# Autodesk Inventor assembly: Intake new robot
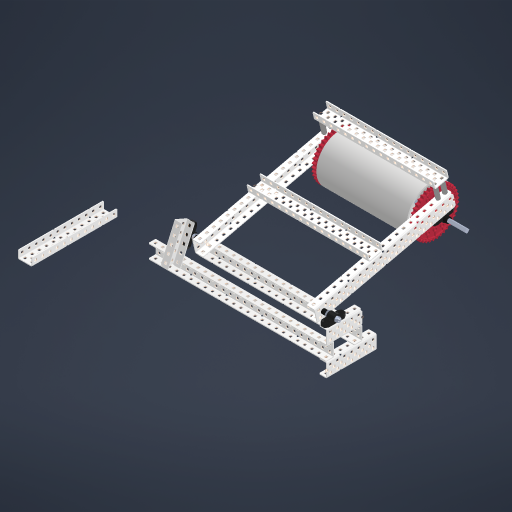
[picture p0: Inventor's stored thumbnail of the model, 512x512]
Saved by Autodesk Inventor 2023.4 (Build 274418000, 418)
## iProperties
Created: 2023-12-04
Part Number: Intake new robot
Document SubType Name: Assembly
Designer: diego
Author: diego
## Documents named in this file (26)
- C:\Users\diego\OneDrive\Documents\GitHub\2024-599Z\2024-599Z\Cad\Intake new robot.iam
- C:\Users\diego\OneDrive\Documents\GitHub\2024-599Z\2024-599Z\Cad\VEX-CAD-Inventor-1.4.0\Structure\C Channel\Aluminum 1x2x1\Alu C 1x2x1x20.ipt
- C:\Users\diego\OneDrive\Documents\GitHub\2024-599Z\2024-599Z\Cad\VEX-CAD-Inventor-1.4.0\Structure\C Channel\Aluminum 1x2x1\Alu C 1x2x1x5.ipt
- C:\Users\diego\OneDrive\Documents\GitHub\2024-599Z\2024-599Z\Cad\VEX-CAD-Inventor-1.4.0\Motion\Shaft HS\HS Pillow Bearing Block.ipt
- C:\Users\diego\OneDrive\Documents\GitHub\2024-599Z\2024-599Z\Cad\VEX-CAD-Inventor-1.4.0\Motion\Spacers\Spacer Plastic.ipt
- C:\Users\diego\OneDrive\Documents\GitHub\2024-599Z\2024-599Z\Cad\VEX-CAD-Inventor-1.4.0\Structure\Hardware\Nut Keps.ipt
- C:\Users\diego\OneDrive\Documents\GitHub\2024-599Z\2024-599Z\Cad\VEX-CAD-Inventor-1.4.0\Structure\Hardware\Screw Steel - Star\SScrew Star Smooth 1.250.ipt
- C:\Users\diego\OneDrive\Documents\GitHub\2024-599Z\2024-599Z\Cad\VEX-CAD-Inventor-1.4.0\Structure\Hardware\Screw Steel - Star.ipt
- C:\Users\diego\OneDrive\Documents\GitHub\2024-599Z\2024-599Z\Cad\VEX-CAD-Inventor-1.4.0\Structure\C Channel\Aluminum 1x2x1\Alu C 1x2x1x1.ipt
- C:\Users\diego\OneDrive\Documents\GitHub\2024-599Z\2024-599Z\Cad\VEX-CAD-Inventor-1.4.0\Structure\Hardware\Nut Nylock_CPY_MIR.ipt
- C:\Users\diego\OneDrive\Documents\GitHub\2024-599Z\2024-599Z\Cad\VEX-CAD-Inventor-1.4.0\Motion\Shaft HS\Shaft HS.ipt
- C:\Users\diego\OneDrive\Documents\GitHub\2024-599Z\2024-599Z\Cad\VEX-CAD-Inventor-1.4.0\Motion\Shaft HS\HS Spacer\HSpacer .0625.ipt
- C:\Users\diego\OneDrive\Documents\GitHub\2024-599Z\2024-599Z\Cad\VEX-CAD-Inventor-1.4.0\Motion\Shaft HS\HS Spacer.ipt
- C:\Users\diego\OneDrive\Documents\GitHub\2024-599Z\2024-599Z\Cad\VEX-CAD-Inventor-1.4.0\Motion\Sprockets\6P Sprocket\6P 40T Sprocket, No Insert.iam
- C:\Users\diego\OneDrive\Documents\GitHub\2024-599Z\2024-599Z\Cad\VEX-CAD-Inventor-1.4.0\Motion\Sprockets\6P Sprocket.iam
- C:\Users\diego\OneDrive\Documents\GitHub\2024-599Z\2024-599Z\Cad\VEX-CAD-Inventor-1.4.0\Motion\Shaft HS\Shaft HS\Shaft HS 10.0 in.ipt
- C:\Users\diego\OneDrive\Documents\GitHub\2024-599Z\2024-599Z\Cad\VEX-CAD-Inventor-1.4.0\Structure\C Channel\Aluminum 1x2x1\Alu C 1x2x1x17.ipt
- C:\Users\diego\OneDrive\Documents\GitHub\2024-599Z\2024-599Z\Cad\VEX-CAD-Inventor-1.4.0\Structure\Standoff\Standoff 1.00.ipt
- C:\Users\Robodox\Documents\GitHub\2024-599Z\Cad\VEX-CAD-Inventor-1.4.0\Structure\Standoff.ipt
- C:\Users\diego\OneDrive\Documents\GitHub\2024-599Z\2024-599Z\Cad\VEX-CAD-Inventor-1.4.0\Structure\C Channel\Aluminum 1x2x1\Alu C 1x2x1x12.ipt
- C:\Users\diego\OneDrive\Documents\GitHub\2024-599Z\2024-599Z\Cad\VEX-CAD-Inventor-1.4.0\Structure\C Channel\Aluminum 1x2x1\Alu C 1x2x1x25.ipt
- C:\Users\diego\OneDrive\Documents\GitHub\2024-599Z\2024-599Z\Cad\VEX-CAD-Inventor-1.4.0\Motion\Spacers\Spacer Plastic\PSpacer 8.0.ipt
- C:\Users\diego\OneDrive\Documents\GitHub\2024-599Z\2024-599Z\Cad\VEX-CAD-Inventor-1.4.0\Structure\C Channel\Aluminum 1x2x1\Alu C 1x2x1x7.ipt
- C:\Users\diego\OneDrive\Documents\GitHub\2024-599Z\2024-599Z\Cad\VEX-CAD-Inventor-1.4.0\Structure\C Channel\Aluminum 1x2x1\Alu C 1x2x1x22.ipt
- C:\Users\diego\OneDrive\Documents\GitHub\2024-599Z\2024-599Z\Cad\mesh intake part.ipt
- C:\Users\diego\OneDrive\Documents\GitHub\2024-599Z\2024-599Z\Cad\VEX-CAD-Inventor-1.4.0\Motion\Shaft HS\HS Spacer\HSpacer .2500.ipt
## Components (37 placed, 19 different names)
1. Alu C 1x2x1x20:1 — Insert:9, Insert:17, Insert:18, Insert:23, Insert:24, Insert:31, Insert:46
2. Alu C 1x2x1x20:2 — Insert:5, Insert:15, Insert:16, Insert:25, Insert:26, Insert:35, Insert:44, Insert:45
3. Alu C 1x2x1x5:1 — Insert:3, Insert:4, Insert:38, Insert:41
4. Alu C 1x2x1x5:2 — Insert:1, Insert:2
5. HS Pillow Bearing Block:1 — Insert:1, Insert:2, Mate:1, Mate:2
6. HS Pillow Bearing Block:2 — Insert:3, Insert:4, Mate:3, Mate:4
7. Nut Keps:1 — Insert:32
8. Nut Keps:2 — Insert:36
9. SScrew Star Smooth 1.250:1 — Insert:9, Insert:14, Insert:33
10. SScrew Star Smooth 1.250:2 — Insert:5, Insert:12, Insert:37
11. HS Pillow Bearing Block:3 — Insert:17, Insert:18, Mate:16, Mate:27, Mate:28, Mate:29, Mate:34, Mate:35
12. HS Pillow Bearing Block:4 — Insert:15, Insert:16, Mate:14, Mate:18, Mate:31, Mate:32, Mate:33
13. Alu C 1x2x1x1:1 — Mate:3, Mate:4, Insert:33
14. Alu C 1x2x1x1:2 — Mate:1, Mate:2, Insert:37
15. Nut Nylock_CPY_MIR:1 — Insert:12
16. Nut Nylock_CPY_MIR:2 — Insert:14
17. HSpacer .0625:1 — Mate:15, Mate:16
18. HSpacer .0625:2 — Mate:12, Mate:13, Mate:14
19. 6P 40T Sprocket, No Insert:1 [sub-assembly] — Mate:26, Mate:27, Insert:47
20. 6P 40T Sprocket, No Insert:2 [sub-assembly] — Mate:30, Mate:31
21. Shaft HS 10.0 in:2 — Mate:12, Mate:13, Mate:15, Mate:18, Mate:26, Mate:30
22. Alu C 1x2x1x17:1 — Insert:27, Insert:28, Insert:29, Mate:17
23. Standoff 1.00:1 — Insert:24, Mate:17
24. Standoff 1.00:2 — Insert:25, Insert:28
25. Standoff 1.00:3 — Insert:23, Insert:29
26. Standoff 1.00:4 — Insert:26, Insert:27
27. Alu C 1x2x1x12:1
28. Alu C 1x2x1x25:1 — Insert:38, Insert:39
29. PSpacer 8.0:3 — Insert:31, Insert:32
30. PSpacer 8.0:4 — Insert:35, Insert:36
31. Alu C 1x2x1x7:1 — Insert:39, Insert:40
32. Alu C 1x2x1x22:1 — Insert:40, Insert:41
33. Alu C 1x2x1x17:2 — Insert:44, Insert:45, Insert:46
34. HSpacer .0625:4 — Mate:28, Mate:29
35. HSpacer .0625:5 — Mate:32, Mate:33
36. mesh intake part:1 — Insert:47
37. HSpacer .2500:6 — Mate:34, Mate:35
## Relationships (54: Insert 33, Mate 21)
- Insert:1: Alu C 1x2x1x5:2 ↔ HS Pillow Bearing Block:1
- Insert:2: Alu C 1x2x1x5:2 ↔ HS Pillow Bearing Block:1
- Insert:3: Alu C 1x2x1x5:1 ↔ HS Pillow Bearing Block:2
- Insert:4: Alu C 1x2x1x5:1 ↔ HS Pillow Bearing Block:2
- Insert:5: Alu C 1x2x1x20:2 ↔ SScrew Star Smooth 1.250:2
- Insert:9: Alu C 1x2x1x20:1 ↔ SScrew Star Smooth 1.250:1
- Mate:1: HS Pillow Bearing Block:1 ↔ Alu C 1x2x1x1:2
- Mate:2: HS Pillow Bearing Block:1 ↔ Alu C 1x2x1x1:2
- Insert:12 (-5.969 mm): SScrew Star Smooth 1.250:2 ↔ Nut Nylock_CPY_MIR:1
- Mate:3: HS Pillow Bearing Block:2 ↔ Alu C 1x2x1x1:1
- Mate:4: HS Pillow Bearing Block:2 ↔ Alu C 1x2x1x1:1
- Insert:14 (-6.096 mm): SScrew Star Smooth 1.250:1 ↔ Nut Nylock_CPY_MIR:2
- Insert:15: Alu C 1x2x1x20:2 ↔ HS Pillow Bearing Block:4
- Insert:16: Alu C 1x2x1x20:2 ↔ HS Pillow Bearing Block:4
- Insert:17: Alu C 1x2x1x20:1 ↔ HS Pillow Bearing Block:3
- Insert:18: Alu C 1x2x1x20:1 ↔ HS Pillow Bearing Block:3
- Mate:12: HSpacer .0625:2 ↔ Shaft HS 10.0 in:2
- Mate:13: HSpacer .0625:2 ↔ Shaft HS 10.0 in:2
- Mate:14: HS Pillow Bearing Block:4 ↔ HSpacer .0625:2
- Mate:15: HSpacer .0625:1 ↔ Shaft HS 10.0 in:2
- Mate:16: HS Pillow Bearing Block:3 ↔ HSpacer .0625:1
- Insert:23: Alu C 1x2x1x20:1 ↔ Standoff 1.00:3
- Insert:24: Alu C 1x2x1x20:1 ↔ Standoff 1.00:1
- Insert:25: Alu C 1x2x1x20:2 ↔ Standoff 1.00:2
- Insert:26: Alu C 1x2x1x20:2 ↔ Standoff 1.00:4
- Insert:27: Alu C 1x2x1x17:1 ↔ Standoff 1.00:4
- Insert:28: Alu C 1x2x1x17:1 ↔ Standoff 1.00:2
- Insert:29: Alu C 1x2x1x17:1 ↔ Standoff 1.00:3
- Mate:17: Alu C 1x2x1x17:1 ↔ Standoff 1.00:1
- Mate:18: HS Pillow Bearing Block:4 ↔ Shaft HS 10.0 in:2
- Insert:31: Alu C 1x2x1x20:1 ↔ PSpacer 8.0:3
- Insert:32: Nut Keps:1 ↔ PSpacer 8.0:3
- Insert:33 (-19.939 mm): SScrew Star Smooth 1.250:1 ↔ Alu C 1x2x1x1:1
- Insert:35: Alu C 1x2x1x20:2 ↔ PSpacer 8.0:4
- Insert:36: Nut Keps:2 ↔ PSpacer 8.0:4
- Insert:37 (-20.066 mm): SScrew Star Smooth 1.250:2 ↔ Alu C 1x2x1x1:2
- Insert:38: Alu C 1x2x1x5:1 ↔ Alu C 1x2x1x25:1
- Insert:39: Alu C 1x2x1x25:1 ↔ Alu C 1x2x1x7:1
- Insert:40: Alu C 1x2x1x7:1 ↔ Alu C 1x2x1x22:1
- Insert:41: Alu C 1x2x1x5:1 ↔ Alu C 1x2x1x22:1
- Insert:44: Alu C 1x2x1x20:2 ↔ Alu C 1x2x1x17:2
- Insert:45: Alu C 1x2x1x20:2 ↔ Alu C 1x2x1x17:2
- Insert:46: Alu C 1x2x1x20:1 ↔ Alu C 1x2x1x17:2
- Mate:26: 6P 40T Sprocket, No Insert:1 ↔ Shaft HS 10.0 in:2
- Mate:27 (1.5875 mm): HS Pillow Bearing Block:3 ↔ 6P 40T Sprocket, No Insert:1
- Mate:28: HS Pillow Bearing Block:3 ↔ HSpacer .0625:4
- Mate:29: HS Pillow Bearing Block:3 ↔ HSpacer .0625:4
- Mate:30: 6P 40T Sprocket, No Insert:2 ↔ Shaft HS 10.0 in:2
- Mate:31 (1.5875 mm): HS Pillow Bearing Block:4 ↔ 6P 40T Sprocket, No Insert:2
- Mate:32: HS Pillow Bearing Block:4 ↔ HSpacer .0625:5
- Mate:33: HS Pillow Bearing Block:4 ↔ HSpacer .0625:5
- Insert:47: 6P 40T Sprocket, No Insert:1 ↔ mesh intake part:1
- Mate:34: HS Pillow Bearing Block:3 ↔ HSpacer .2500:6
- Mate:35: HS Pillow Bearing Block:3 ↔ HSpacer .2500:6
